# Autodesk Inventor assembly: Crank
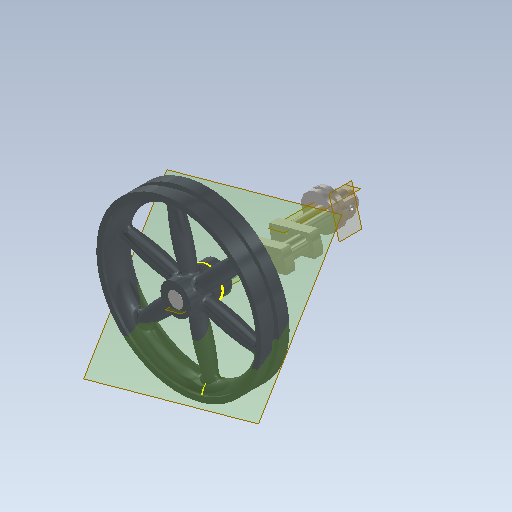
[picture p0: Inventor's stored thumbnail of the model, 512x512]
Saved by Autodesk Inventor 2020 (Build 240168000, 168)
## iProperties
Created: 2021-10-25
Part Number: Crank
Document SubType Name: Assembly
Designer: simon.erikssonwestl
Author: simon.erikssonwestl
## Documents named in this file (10)
- C:\Users\simon.erikssonwestl\Documents\Inventor\Ång\Assemblies\Crank.iam
- C:\Users\simon.erikssonwestl\Documents\Inventor\Ång\Part18.ipt
- C:\Users\simon.erikssonwestl\Documents\Inventor\Ång\Part13.ipt
- C:\Users\simon.erikssonwestl\Documents\Inventor\Ång\Part16.ipt
- C:\Users\simon.erikssonwestl\Documents\Inventor\Ång\Part14.ipt
- C:\Users\simon.erikssonwestl\Documents\Inventor\Ång\Part15.ipt
- C:\Users\simon.erikssonwestl\Documents\Inventor\Ång\Part12.ipt
- C:\Users\simon.erikssonwestl\Documents\Inventor\Ång\Part17.ipt
- C:\Users\simon.erikssonwestl\Documents\Inventor\Content Center Files\R2020\en-US\AS 1421(2)\AS 1421 - M3 x 4 Cup Point.ipt
- C:\Users\simon.erikssonwestl\Documents\Inventor\Content Center Files\R2020\en-US\ANSI B18.3.6M(01)\ANSI B18.3.6M - M2,5x0,45 x 2,5(2).ipt
## Components (11 placed, 9 different names)
1. Part18:1 — Mate:1, Angle:1, Flush:1, Mate:11
2. Part13:1 — Mate:1, Angle:1, Flush:1, Mate:2, Mate:4, Flush:2, Angle:2, Mate:9, Angle:3, Tangent:1
3. Part16:1 — Mate:2, Flush:3
4. Part14:1 — Mate:4, Flush:2, Angle:2, Flush:3, Mate:5, Flush:4
5. Part15:1 — Mate:5, Flush:4, Mate:6, Flush:6
6. Part14:2 — Mate:6, Mate:7, Flush:5, Flush:6, Mate:8, Flush:7
7. Part16:2 — Mate:7, Flush:5
8. Part12:1 — Mate:8, Mate:9, Flush:7, Mate:10, Tangent:2
9. Part17:1 — Mate:10, Angle:3, Mate:12
10. AS 1421 Cup Point - Metric M3 x 4 Cup Point:1 — Mate:11, Tangent:1
11. Broached Hexagon Socket Set Screw - Flat Point - Metric M2,5x0,45 x 2,5:1 — Mate:12, Tangent:2
## Relationships (23: Mate 11, Flush 7, Angle 3, Tangent 2)
- Mate:1: Part18:1 ↔ Part13:1
- Angle:1 (90 deg): Part18:1 ↔ Part13:1
- Flush:1: Part18:1 ↔ Part13:1
- Mate:2: Part13:1 ↔ Part16:1
- Mate:4: Part13:1 ↔ Part14:1
- Flush:2: Part13:1 ↔ Part14:1
- Angle:2 (180 deg): Part13:1 ↔ Part14:1
- Flush:3: Part16:1 ↔ Part14:1
- Mate:5: Part14:1 ↔ Part15:1
- Flush:4: Part14:1 ↔ Part15:1
- Mate:6: Part15:1 ↔ Part14:2
- Mate:7: Part14:2 ↔ Part16:2
- Flush:5: Part14:2 ↔ Part16:2
- Flush:6: Part15:1 ↔ Part14:2
- Mate:8: Part14:2 ↔ Part12:1
- Mate:9: Part13:1 ↔ Part12:1
- Flush:7: Part14:2 ↔ Part12:1
- Mate:10: Part12:1 ↔ Part17:1
- Angle:3 (-90 deg): Part13:1 ↔ Part17:1
- Mate:11: Part18:1 ↔ AS 1421 Cup Point - Metric M3 x 4 Cup Point:1
- Tangent:1: Part13:1 ↔ AS 1421 Cup Point - Metric M3 x 4 Cup Point:1
- Mate:12: Part17:1 ↔ Broached Hexagon Socket Set Screw - Flat Point - Metric M2,5x0,45 x 2,5:1
- Tangent:2: Part12:1 ↔ Broached Hexagon Socket Set Screw - Flat Point - Metric M2,5x0,45 x 2,5:1
